# Autodesk Inventor assembly: hw2
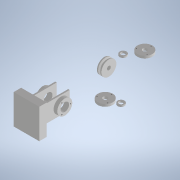
[picture p0: Inventor's stored thumbnail of the model, 180x180]
Saved by Autodesk Inventor 2020 (Build 240168000, 168)
## iProperties
Created: 2021-12-07
Part Number: hw2
Document SubType Name: Assembly
Designer: Umur Batuhan Özmen
Author: Umur Batuhan Özmen
## Documents named in this file (6)
- C:\Users\umuro\OneDrive - ikc.edu.tr\Home - Library_Umur\E\Education\2020-2024_Mechatronics\Lessons\MEE203-DINAMIK\Whales_Dynamics_Project\Drawings\hw2.iam
- C:\Users\umuro\OneDrive - ikc.edu.tr\Home - Library_Umur\E\Education\2020-2024_Mechatronics\Lessons\MEE112-BILGISAYAR_DESTEKLI_TEKNIK_RESIM_II\Drawings\hw2\Base.ipt
- C:\Users\umuro\OneDrive - ikc.edu.tr\Home - Library_Umur\E\Education\2020-2024_Mechatronics\Lessons\MEE112-BILGISAYAR_DESTEKLI_TEKNIK_RESIM_II\Drawings\hw2\Housing.ipt
- C:\Users\umuro\OneDrive - ikc.edu.tr\Home - Library_Umur\E\Education\2020-2024_Mechatronics\Lessons\MEE112-BILGISAYAR_DESTEKLI_TEKNIK_RESIM_II\Drawings\hw2\Pulley.ipt
- C:\Users\umuro\OneDrive - ikc.edu.tr\Home - Library_Umur\E\Education\2020-2024_Mechatronics\Lessons\MEE112-BILGISAYAR_DESTEKLI_TEKNIK_RESIM_II\Drawings\hw2\Seal.ipt
- C:\Users\umuro\OneDrive - ikc.edu.tr\Home - Library_Umur\E\Education\2020-2024_Mechatronics\Lessons\MEE112-BILGISAYAR_DESTEKLI_TEKNIK_RESIM_II\Drawings\hw2\Seal_Cover.ipt
## Components (7 placed, 5 different names)
1. Base:1 — Mate:1, Mate:2, Mate:3
2. Housing:1 — Mate:1, Mate:2, Mate:3
3. Pulley:1
4. Seal:1
5. Seal_Cover:1
6. Seal:2
7. Seal_Cover:2
## Relationships (3: Mate 3)
- Mate:1: Base:1 ↔ Housing:1
- Mate:2: Base:1 ↔ Housing:1
- Mate:3: Base:1 ↔ Housing:1
